# Autodesk Inventor assembly: leg_1
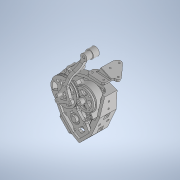
[picture p0: Inventor's stored thumbnail of the model, 180x180]
Saved by Autodesk Inventor 2020 (Build 240168000, 168)
## iProperties
Created: 2020-12-08
Part Number: leg_1
Document SubType Name: Assembly
Designer: Shuang Peng
Author: Shuang Peng
## Documents named in this file (11)
- D:\projects-3\biped_tiny\hardware\sim_mod\leg_1_sim.iam
- D:\projects-3\biped_tiny\hardware\sim_mod\reducer_1.iam
- D:\projects-3\biped_tiny\hardware\leg_holder_2.ipt
- D:\projects-3\biped_tiny\hardware\leg_link_1.ipt
- D:\projects-3\biped_tiny\hardware\leg_link_2.ipt
- D:\projects-3\biped_tiny\hardware\leg_link_4.ipt
- D:\projects-3\biped_tiny\hardware\leg_link_3_m.ipt
- D:\projects-3\biped_tiny\hardware\foot_2.ipt
- D:\projects-3\biped_tiny\hardware\pin_3_15.ipt
- D:\projects-3\biped_tiny\hardware\body_conn_1.ipt
- D:\projects-3\biped_tiny\hardware\body_conn_2.ipt
## Components (16 placed, 10 different names)
1. reducer_1:1 [sub-assembly] — Insert:42, Insert:43, Insert:46
2. leg_holder_2:1 — Insert:40, Insert:41, Insert:42, Insert:43, Insert:44, Insert:45, Insert:49, Insert:50, Angle:1, Angle:2
3. leg_link_1:1 — Flush:5, Flush:6, Insert:9, Insert:16, Flush:7, Insert:18, Insert:19
4. leg_link_2:1 — Flush:6, Insert:9, Insert:26, Insert:47, Angle:1, Insert:51
5. leg_link_4:1 — Insert:17, Insert:46, Angle:2, Insert:52
6. leg_link_3_m:1 — Insert:16, Insert:17, Insert:27, Insert:28
7. foot_2:1 — Flush:7, Insert:18, Insert:19
8. pin_3_15:1 — Insert:26
9. pin_3_15:2 — Insert:27
10. pin_3_15:3 — Insert:28
11. reducer_1:3 [sub-assembly] — Insert:44, Insert:45, Insert:47
12. body_conn_1:1 — Insert:40, Insert:41, Insert:48
13. pin_3_15:4 — Insert:48
14. body_conn_2:1 — Insert:49, Insert:50
15. pin_3_15:5 — Insert:51
16. pin_3_15:6 — Insert:52
## Relationships (26: Insert 21, Flush 3, Angle 2)
- Flush:5: leg_link_1:1
- Flush:6: leg_link_1:1 ↔ leg_link_2:1
- Insert:9: leg_link_1:1 ↔ leg_link_2:1
- Insert:16: leg_link_1:1 ↔ leg_link_3_m:1
- Insert:17: leg_link_4:1 ↔ leg_link_3_m:1
- Flush:7: leg_link_1:1 ↔ foot_2:1
- Insert:18: leg_link_1:1 ↔ foot_2:1
- Insert:19: leg_link_1:1 ↔ foot_2:1
- Insert:26: leg_link_2:1 ↔ pin_3_15:1
- Insert:27: leg_link_3_m:1 ↔ pin_3_15:2
- Insert:28: leg_link_3_m:1 ↔ pin_3_15:3
- Insert:40: leg_holder_2:1 ↔ body_conn_1:1
- Insert:41: leg_holder_2:1 ↔ body_conn_1:1
- Insert:42: reducer_1:1 ↔ leg_holder_2:1
- Insert:43: reducer_1:1 ↔ leg_holder_2:1
- Insert:44: leg_holder_2:1 ↔ reducer_1:3
- Insert:45: leg_holder_2:1 ↔ reducer_1:3
- Insert:46: reducer_1:1 ↔ leg_link_4:1
- Insert:47: leg_link_2:1 ↔ reducer_1:3
- Insert:48 (-12 mm): body_conn_1:1 ↔ pin_3_15:4
- Insert:49: leg_holder_2:1 ↔ body_conn_2:1
- Insert:50: leg_holder_2:1 ↔ body_conn_2:1
- Angle:1 (0 deg): leg_holder_2:1 ↔ leg_link_2:1
- Angle:2 (0 deg): leg_holder_2:1 ↔ leg_link_4:1
- Insert:51 (-5 mm): leg_link_2:1 ↔ pin_3_15:5
- Insert:52 (-5 mm): leg_link_4:1 ↔ pin_3_15:6
